# Autodesk Inventor assembly: auger_assembly
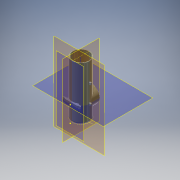
[picture p0: Inventor's stored thumbnail of the model, 180x180]
Saved by Autodesk Inventor 2019 (Build 230136000, 136)
## iProperties
Created: 2019-05-05
Part Number: auger_assembly
Document SubType Name: Assembly
Designer: assman
Author: assman
## Documents named in this file (3)
- D:\Inventor\Projects\CatFeeder\Case\version7\auger_assembly.iam
- D:\Inventor\Projects\CatFeeder\Case\version7\auger_case.ipt
- D:\Inventor\Projects\CatFeeder\Case\version7\auger.ipt
## Components (2 placed, 2 different names)
1. auger_case:1 — Flush:1, Flush:2, Flush:3
2. auger:1 — Flush:1, Flush:2
## Relationships (3: Flush 3)
- Flush:1: auger_case:1 ↔ auger:1
- Flush:2: auger_case:1 ↔ auger:1
- Flush:3: auger_case:1
